# Autodesk Inventor assembly: WelcoMount_wSwitch
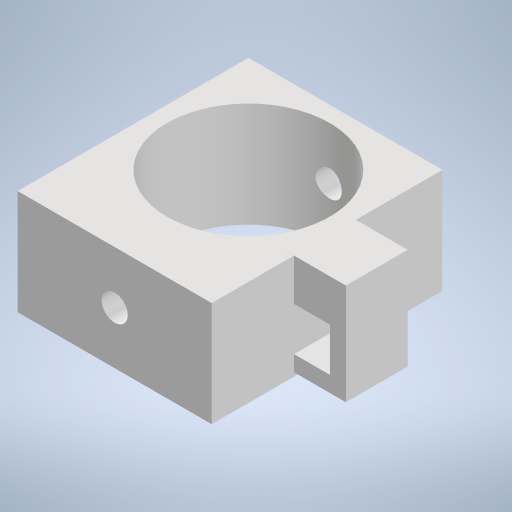
[picture p0: Inventor's stored thumbnail of the model, 512x512]
Saved by Autodesk Inventor 2023.5 (Build 275446000, 446)
## iProperties
Created: 2024-08-19
Part Number: WelcoMount_wSwitch
Document SubType Name: Assembly
Designer: Akramilab
Author: Akramilab
## Documents named in this file (3)
- C:\Projects\Inventor\Touchscreen arena\Welco pump mount\WelcoMount_wSwitch.iam
- C:\Projects\Inventor\Touchscreen arena\Welco pump mount\switch test v02b.ipt
- C:\Projects\Inventor\Touchscreen arena\Welco pump mount\welco mount v03.ipt
## Components (2 placed, 2 different names)
1. welco mount v03:1 — Flush:1, Flush:2, Mate:1, Flush:3
2. switch test v02b:1 — Flush:1, Flush:2, Mate:1, Flush:3
## Relationships (4: Flush 3, Mate 1)
- Flush:1 (16.51 mm): welco mount v03:1 ↔ switch test v02b:1
- Flush:2: welco mount v03:1 ↔ switch test v02b:1
- Mate:1 (-3 mm): welco mount v03:1 ↔ switch test v02b:1
- Flush:3: welco mount v03:1 ↔ switch test v02b:1
